# Autodesk Inventor assembly: assembly
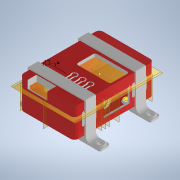
[picture p0: Inventor's stored thumbnail of the model, 180x180]
Saved by Autodesk Inventor 2020 (Build 240168000, 168)
## iProperties
Created: 2019-09-23
Part Number: assembly
Document SubType Name: Assembly
Designer: erwin
Author: erwin
## Documents named in this file (4)
- D:\GitHub\ElCheapoAIS-nmea\case\OrangeZero\source-ttgoterm\assembly.iam
- D:\GitHub\ElCheapoAIS-nmea\case\OrangeZero\source\bottom_part.ipt
- D:\GitHub\ElCheapoAIS-nmea\case\OrangeZero\source-ttgoterm\top_lcd.ipt
- D:\GitHub\ElCheapoAIS-nmea\case\OrangeZero\source\rail_clip.ipt
## Components (4 placed, 3 different names)
1. bottom_part:1 — Flush:2, Flush:3, Mate:1, Mate:4, Mate:6, Mate:7
2. top_lcd:1 — Flush:2, Flush:3, Mate:1, Mate:2, Mate:3, Mate:5
3. rail_clip:1 — Mate:2, Mate:4, Mate:7
4. rail_clip:2 — Mate:3, Mate:5, Mate:6
## Relationships (9: Mate 7, Flush 2)
- Flush:2: bottom_part:1 ↔ top_lcd:1
- Flush:3: bottom_part:1 ↔ top_lcd:1
- Mate:1: bottom_part:1 ↔ top_lcd:1
- Mate:2: top_lcd:1 ↔ rail_clip:1
- Mate:3: top_lcd:1 ↔ rail_clip:2
- Mate:4: bottom_part:1 ↔ rail_clip:1
- Mate:5: top_lcd:1 ↔ rail_clip:2
- Mate:6: bottom_part:1 ↔ rail_clip:2
- Mate:7: bottom_part:1 ↔ rail_clip:1
